# Autodesk Inventor assembly: SACMI DPA CARDBOARD POSITIONING SYSMEM
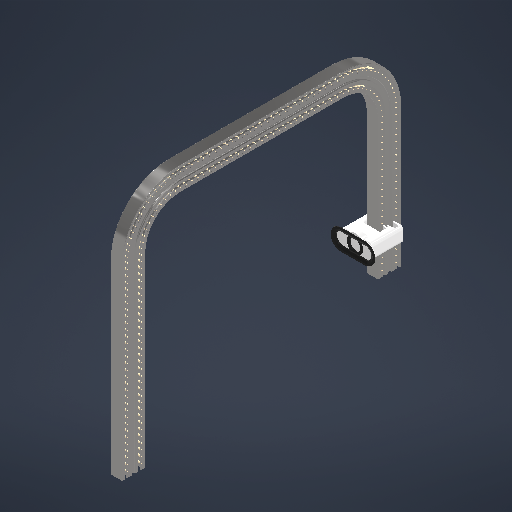
[picture p0: Inventor's stored thumbnail of the model, 512x512]
Saved by Autodesk Inventor 2025 (Build 290162000, 162)
## iProperties
Created: 2024-05-16
Part Number: SACMI DPA CARDBOARD POSITIONING SYSMEM
Document SubType Name: Assembly
Designer: zulet
Author: zulet
## Documents named in this file (4)
- D:\UNAL\2024-1S\APM\Digital Factory\Packaging Machine\SACMI DPA CARDBOARD POSITIONING SYSMEM.iam
- D:\UNAL\2024-1S\APM\Digital Factory\Packaging Machine\SACMI DPA C-RAIL.ipt
- D:\UNAL\2024-1S\APM\Digital Factory\Packaging Machine\SCAMI D-PA C-RAIL ROLLER.ipt
- D:\UNAL\2024-1S\APM\Digital Factory\Packaging Machine\SACMI DPA C-RAIL GRIP.ipt
## Components (226 placed, 3 different names)
1. SACMI DPA C-RAIL:1 — Mate:1, Mate:2, Flush:1, Mate:3, Flush:2
2. SACMI DPA C-RAIL GRIP:1 — Flush:1, Mate:3, Flush:2
3. SCAMI D-PA C-RAIL ROLLER:1 — Mate:1, Mate:2
4. SCAMI D-PA C-RAIL ROLLER:2
5. SCAMI D-PA C-RAIL ROLLER:3
6. SCAMI D-PA C-RAIL ROLLER:4
7. SCAMI D-PA C-RAIL ROLLER:5
8. SCAMI D-PA C-RAIL ROLLER:6
9. SCAMI D-PA C-RAIL ROLLER:7
10. SCAMI D-PA C-RAIL ROLLER:8
11. SCAMI D-PA C-RAIL ROLLER:9
12. SCAMI D-PA C-RAIL ROLLER:10
13. SCAMI D-PA C-RAIL ROLLER:11
14. SCAMI D-PA C-RAIL ROLLER:12
15. SCAMI D-PA C-RAIL ROLLER:13
16. SCAMI D-PA C-RAIL ROLLER:14
17. SCAMI D-PA C-RAIL ROLLER:15
18. SCAMI D-PA C-RAIL ROLLER:16
19. SCAMI D-PA C-RAIL ROLLER:17
20. SCAMI D-PA C-RAIL ROLLER:18
21. SCAMI D-PA C-RAIL ROLLER:19
22. SCAMI D-PA C-RAIL ROLLER:20
23. SCAMI D-PA C-RAIL ROLLER:21
24. SCAMI D-PA C-RAIL ROLLER:22
25. SCAMI D-PA C-RAIL ROLLER:23
26. SCAMI D-PA C-RAIL ROLLER:24
27. SCAMI D-PA C-RAIL ROLLER:25
28. SCAMI D-PA C-RAIL ROLLER:26
29. SCAMI D-PA C-RAIL ROLLER:27
30. SCAMI D-PA C-RAIL ROLLER:28
31. SCAMI D-PA C-RAIL ROLLER:29
32. SCAMI D-PA C-RAIL ROLLER:30
33. SCAMI D-PA C-RAIL ROLLER:31
34. SCAMI D-PA C-RAIL ROLLER:32
35. SCAMI D-PA C-RAIL ROLLER:33
36. SCAMI D-PA C-RAIL ROLLER:34
37. SCAMI D-PA C-RAIL ROLLER:35
38. SCAMI D-PA C-RAIL ROLLER:36
39. SCAMI D-PA C-RAIL ROLLER:37
40. SCAMI D-PA C-RAIL ROLLER:38
41. SCAMI D-PA C-RAIL ROLLER:39
42. SCAMI D-PA C-RAIL ROLLER:40
43. SCAMI D-PA C-RAIL ROLLER:41
44. SCAMI D-PA C-RAIL ROLLER:42
45. SCAMI D-PA C-RAIL ROLLER:43
46. SCAMI D-PA C-RAIL ROLLER:44
47. SCAMI D-PA C-RAIL ROLLER:45
48. SCAMI D-PA C-RAIL ROLLER:46
49. SCAMI D-PA C-RAIL ROLLER:47
50. SCAMI D-PA C-RAIL ROLLER:48
51. SCAMI D-PA C-RAIL ROLLER:49
52. SCAMI D-PA C-RAIL ROLLER:50
53. SCAMI D-PA C-RAIL ROLLER:51
54. SCAMI D-PA C-RAIL ROLLER:52
55. SCAMI D-PA C-RAIL ROLLER:53
56. SCAMI D-PA C-RAIL ROLLER:54
57. SCAMI D-PA C-RAIL ROLLER:55
58. SCAMI D-PA C-RAIL ROLLER:56
59. SCAMI D-PA C-RAIL ROLLER:57
60. SCAMI D-PA C-RAIL ROLLER:58
61. SCAMI D-PA C-RAIL ROLLER:59
62. SCAMI D-PA C-RAIL ROLLER:60
63. SCAMI D-PA C-RAIL ROLLER:61
64. SCAMI D-PA C-RAIL ROLLER:62
65. SCAMI D-PA C-RAIL ROLLER:63
66. SCAMI D-PA C-RAIL ROLLER:64
67. SCAMI D-PA C-RAIL ROLLER:65
68. SCAMI D-PA C-RAIL ROLLER:66
69. SCAMI D-PA C-RAIL ROLLER:67
70. SCAMI D-PA C-RAIL ROLLER:68
71. SCAMI D-PA C-RAIL ROLLER:69
72. SCAMI D-PA C-RAIL ROLLER:70
73. SCAMI D-PA C-RAIL ROLLER:71
74. SCAMI D-PA C-RAIL ROLLER:72
75. SCAMI D-PA C-RAIL ROLLER:73
76. SCAMI D-PA C-RAIL ROLLER:74
77. SCAMI D-PA C-RAIL ROLLER:75
78. SCAMI D-PA C-RAIL ROLLER:76
79. SCAMI D-PA C-RAIL ROLLER:77
80. SCAMI D-PA C-RAIL ROLLER:78
81. SCAMI D-PA C-RAIL ROLLER:79
82. SCAMI D-PA C-RAIL ROLLER:80
83. SCAMI D-PA C-RAIL ROLLER:81
84. SCAMI D-PA C-RAIL ROLLER:82
85. SCAMI D-PA C-RAIL ROLLER:83
86. SCAMI D-PA C-RAIL ROLLER:84
87. SCAMI D-PA C-RAIL ROLLER:85
88. SCAMI D-PA C-RAIL ROLLER:86
89. SCAMI D-PA C-RAIL ROLLER:87
90. SCAMI D-PA C-RAIL ROLLER:88
91. SCAMI D-PA C-RAIL ROLLER:89
92. SCAMI D-PA C-RAIL ROLLER:90
93. SCAMI D-PA C-RAIL ROLLER:91
94. SCAMI D-PA C-RAIL ROLLER:92
95. SCAMI D-PA C-RAIL ROLLER:93
96. SCAMI D-PA C-RAIL ROLLER:94
97. SCAMI D-PA C-RAIL ROLLER:95
98. SCAMI D-PA C-RAIL ROLLER:96
99. SCAMI D-PA C-RAIL ROLLER:97
100. SCAMI D-PA C-RAIL ROLLER:98
101. SCAMI D-PA C-RAIL ROLLER:99
102. SCAMI D-PA C-RAIL ROLLER:100
103. SCAMI D-PA C-RAIL ROLLER:101
104. SCAMI D-PA C-RAIL ROLLER:102
105. SCAMI D-PA C-RAIL ROLLER:103
106. SCAMI D-PA C-RAIL ROLLER:104
107. SCAMI D-PA C-RAIL ROLLER:105
108. SCAMI D-PA C-RAIL ROLLER:106
109. SCAMI D-PA C-RAIL ROLLER:107
110. SCAMI D-PA C-RAIL ROLLER:108
111. SCAMI D-PA C-RAIL ROLLER:109
112. SCAMI D-PA C-RAIL ROLLER:110
113. SCAMI D-PA C-RAIL ROLLER:111
114. SCAMI D-PA C-RAIL ROLLER:112
115. SCAMI D-PA C-RAIL ROLLER:113
116. SCAMI D-PA C-RAIL ROLLER:114
117. SCAMI D-PA C-RAIL ROLLER:115
118. SCAMI D-PA C-RAIL ROLLER:116
119. SCAMI D-PA C-RAIL ROLLER:117
120. SCAMI D-PA C-RAIL ROLLER:118
121. SCAMI D-PA C-RAIL ROLLER:119
122. SCAMI D-PA C-RAIL ROLLER:120
123. SCAMI D-PA C-RAIL ROLLER:121
124. SCAMI D-PA C-RAIL ROLLER:122
125. SCAMI D-PA C-RAIL ROLLER:123
126. SCAMI D-PA C-RAIL ROLLER:124
127. SCAMI D-PA C-RAIL ROLLER:125
128. SCAMI D-PA C-RAIL ROLLER:126
129. SCAMI D-PA C-RAIL ROLLER:127
130. SCAMI D-PA C-RAIL ROLLER:128
131. SCAMI D-PA C-RAIL ROLLER:129
132. SCAMI D-PA C-RAIL ROLLER:130
133. SCAMI D-PA C-RAIL ROLLER:131
134. SCAMI D-PA C-RAIL ROLLER:132
135. SCAMI D-PA C-RAIL ROLLER:133
136. SCAMI D-PA C-RAIL ROLLER:134
137. SCAMI D-PA C-RAIL ROLLER:135
138. SCAMI D-PA C-RAIL ROLLER:136
139. SCAMI D-PA C-RAIL ROLLER:137
140. SCAMI D-PA C-RAIL ROLLER:138
141. SCAMI D-PA C-RAIL ROLLER:139
142. SCAMI D-PA C-RAIL ROLLER:140
143. SCAMI D-PA C-RAIL ROLLER:141
144. SCAMI D-PA C-RAIL ROLLER:142
145. SCAMI D-PA C-RAIL ROLLER:143
146. SCAMI D-PA C-RAIL ROLLER:144
147. SCAMI D-PA C-RAIL ROLLER:145
148. SCAMI D-PA C-RAIL ROLLER:146
149. SCAMI D-PA C-RAIL ROLLER:147
150. SCAMI D-PA C-RAIL ROLLER:148
151. SCAMI D-PA C-RAIL ROLLER:149
152. SCAMI D-PA C-RAIL ROLLER:150
153. SCAMI D-PA C-RAIL ROLLER:151
154. SCAMI D-PA C-RAIL ROLLER:152
155. SCAMI D-PA C-RAIL ROLLER:153
156. SCAMI D-PA C-RAIL ROLLER:154
157. SCAMI D-PA C-RAIL ROLLER:155
158. SCAMI D-PA C-RAIL ROLLER:156
159. SCAMI D-PA C-RAIL ROLLER:157
160. SCAMI D-PA C-RAIL ROLLER:158
161. SCAMI D-PA C-RAIL ROLLER:159
162. SCAMI D-PA C-RAIL ROLLER:160
163. SCAMI D-PA C-RAIL ROLLER:161
164. SCAMI D-PA C-RAIL ROLLER:162
165. SCAMI D-PA C-RAIL ROLLER:163
166. SCAMI D-PA C-RAIL ROLLER:164
167. SCAMI D-PA C-RAIL ROLLER:165
168. SCAMI D-PA C-RAIL ROLLER:166
169. SCAMI D-PA C-RAIL ROLLER:167
170. SCAMI D-PA C-RAIL ROLLER:168
171. SCAMI D-PA C-RAIL ROLLER:169
172. SCAMI D-PA C-RAIL ROLLER:170
173. SCAMI D-PA C-RAIL ROLLER:171
174. SCAMI D-PA C-RAIL ROLLER:172
175. SCAMI D-PA C-RAIL ROLLER:173
176. SCAMI D-PA C-RAIL ROLLER:174
177. SCAMI D-PA C-RAIL ROLLER:175
178. SCAMI D-PA C-RAIL ROLLER:176
179. SCAMI D-PA C-RAIL ROLLER:177
180. SCAMI D-PA C-RAIL ROLLER:178
181. SCAMI D-PA C-RAIL ROLLER:179
182. SCAMI D-PA C-RAIL ROLLER:180
183. SCAMI D-PA C-RAIL ROLLER:181
184. SCAMI D-PA C-RAIL ROLLER:182
185. SCAMI D-PA C-RAIL ROLLER:183
186. SCAMI D-PA C-RAIL ROLLER:184
187. SCAMI D-PA C-RAIL ROLLER:185
188. SCAMI D-PA C-RAIL ROLLER:186
189. SCAMI D-PA C-RAIL ROLLER:187
190. SCAMI D-PA C-RAIL ROLLER:188
191. SCAMI D-PA C-RAIL ROLLER:189
192. SCAMI D-PA C-RAIL ROLLER:190
193. SCAMI D-PA C-RAIL ROLLER:191
194. SCAMI D-PA C-RAIL ROLLER:192
195. SCAMI D-PA C-RAIL ROLLER:193
196. SCAMI D-PA C-RAIL ROLLER:194
197. SCAMI D-PA C-RAIL ROLLER:195
198. SCAMI D-PA C-RAIL ROLLER:196
199. SCAMI D-PA C-RAIL ROLLER:197
200. SCAMI D-PA C-RAIL ROLLER:198
201. SCAMI D-PA C-RAIL ROLLER:199
202. SCAMI D-PA C-RAIL ROLLER:200
203. SCAMI D-PA C-RAIL ROLLER:201
204. SCAMI D-PA C-RAIL ROLLER:202
205. SCAMI D-PA C-RAIL ROLLER:203
206. SCAMI D-PA C-RAIL ROLLER:204
207. SCAMI D-PA C-RAIL ROLLER:205
208. SCAMI D-PA C-RAIL ROLLER:206
209. SCAMI D-PA C-RAIL ROLLER:207
210. SCAMI D-PA C-RAIL ROLLER:208
211. SCAMI D-PA C-RAIL ROLLER:209
212. SCAMI D-PA C-RAIL ROLLER:210
213. SCAMI D-PA C-RAIL ROLLER:211
214. SCAMI D-PA C-RAIL ROLLER:212
215. SCAMI D-PA C-RAIL ROLLER:213
216. SCAMI D-PA C-RAIL ROLLER:214
217. SCAMI D-PA C-RAIL ROLLER:215
218. SCAMI D-PA C-RAIL ROLLER:216
219. SCAMI D-PA C-RAIL ROLLER:217
220. SCAMI D-PA C-RAIL ROLLER:218
221. SCAMI D-PA C-RAIL ROLLER:219
222. SCAMI D-PA C-RAIL ROLLER:220
223. SCAMI D-PA C-RAIL ROLLER:221
224. SCAMI D-PA C-RAIL ROLLER:222
225. SCAMI D-PA C-RAIL ROLLER:223
226. SCAMI D-PA C-RAIL ROLLER:224
## Component patterns: (224 elements, first: SCAMI D-PA C-RAIL ROLLER:1)
## Relationships (5: Mate 3, Flush 2)
- Mate:1: SACMI DPA C-RAIL:1 ↔ SCAMI D-PA C-RAIL ROLLER:1
- Mate:2 (0.25 mm): SACMI DPA C-RAIL:1 ↔ SCAMI D-PA C-RAIL ROLLER:1
- Flush:1 (120 mm): SACMI DPA C-RAIL:1 ↔ SACMI DPA C-RAIL GRIP:1
- Mate:3: SACMI DPA C-RAIL:1 ↔ SACMI DPA C-RAIL GRIP:1
- Flush:2: SACMI DPA C-RAIL:1 ↔ SACMI DPA C-RAIL GRIP:1
